# Autodesk Inventor assembly: Orange_PI_Cover
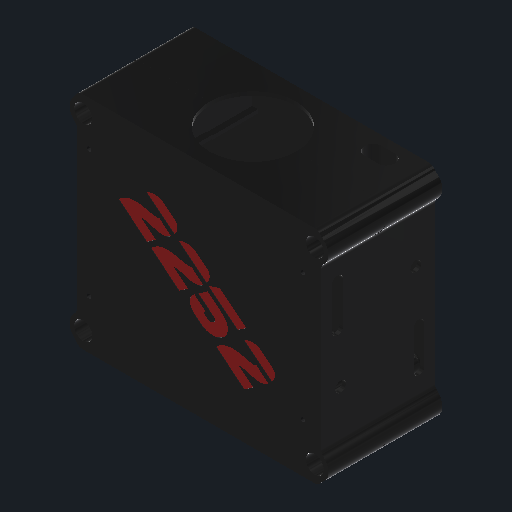
[picture p0: Inventor's stored thumbnail of the model, 512x512]
Saved by Autodesk Inventor 2023 (Build 270158000, 158)
## iProperties
Created: 2024-02-20
Part Number: Orange_PI_Cover
Document SubType Name: Assembly
Designer: mavericks
Author: mavericks
## Documents named in this file (3)
- C:\Users\dlangdon\Documents\GitHub\Crescendo_2024-CAD\2024 Robot\COMMON PARTS\ELECTRONICS\OrangePi\Orange_Pi_Cover_001\Orange_PI_Cover.iam
- C:\Users\dlangdon\Documents\GitHub\Crescendo_2024-CAD\2024 Robot\COMMON PARTS\ELECTRONICS\OrangePi\Orange_Pi_Cover_001\orangepicover-001.ipt
- C:\Users\dlangdon\Documents\GitHub\Crescendo_2024-CAD\2024 Robot\COMMON PARTS\ELECTRONICS\OrangePi\Orange_Pi_Cover_001\orangepicover-001a.ipt
## Components (2 placed, 2 different names)
1. orangepicover-001:1 — Flush:1, Flush:2, Insert:1
2. orangepicover-001a:1 — Flush:1, Flush:2, Insert:1
## Relationships (3: Flush 2, Insert 1)
- Flush:1: orangepicover-001:1 ↔ orangepicover-001a:1
- Flush:2: orangepicover-001:1 ↔ orangepicover-001a:1
- Insert:1: orangepicover-001:1 ↔ orangepicover-001a:1
